# Autodesk Inventor assembly: Clamp-On Single Stage Gearbox
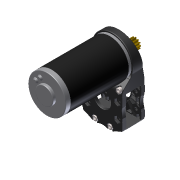
[picture p0: Inventor's stored thumbnail of the model, 180x180]
Saved by Autodesk Inventor 2015 (Build 190159000, 159)
## iProperties
Created: 2014-12-18
Part Number: Clamp-On Single Stage Gearbox
Document SubType Name: Assembly
Designer: Nemo
Author: Nemo
## Documents named in this file (8)
- H:\Nemo\Documents\Robotics\CAD Files\COTS Parts\Gearboxes\VexPro\Clamp-On Single Stage Gearbox.iam
- H:\Nemo\Documents\Robotics\CAD Files\COTS Parts\Gearboxes\VexPro\Components\Clamp-On Single Stage Gearbox motor side.ipt
- H:\Nemo\Documents\Robotics\CAD Files\COTS Parts\Gearboxes\VexPro\Components\Clamp-On Single Stage Gearbox gear side.ipt
- H:\Nemo\Documents\Robotics\CAD Files\COTS Parts\Fasteners\10-32\10-32 locknut.ipt
- H:\Nemo\Documents\Robotics\CAD Files\COTS Parts\Fasteners\10-32\10-32 SHCS x1375.ipt
- H:\Nemo\Documents\Robotics\CAD Files\COTS Parts\Motors\CIM motor.ipt
- H:\Nemo\Documents\Robotics\CAD Files\COTS Parts\Gears\Gear 20dp 10mm key 12T Vex.ipt
- H:\Nemo\Documents\Robotics\CAD Files\COTS Parts\Fasteners\10-32\10-32 SHCS x625.ipt
## Components (14 placed, 7 different names)
1. Clamp-On Single Stage Gearbox motor side:1 — Mate:6, Flush:1, Mate:7, Flush:3, Insert:9, Mate:8, Insert:10, Insert:11, Insert:12, Insert:13, Insert:14, Insert:15, Flush:4
2. Clamp-On Single Stage Gearbox gear side:1 — Insert:5, Insert:6, Insert:7, Insert:8, Mate:6, Flush:2, Mate:7
3. 10-32 locknut:1 — Insert:12
4. 10-32 locknut:2 — Insert:13
5. 10-32 locknut:3 — Insert:14
6. 10-32 locknut:4 — Insert:15
7. 10-32 SHCS x1375:1 — Insert:5
8. 10-32 SHCS x1375:2 — Insert:6
9. 10-32 SHCS x1375:3 — Insert:7
10. 10-32 SHCS x1375:4 — Insert:8
11. CIM motor:1 — Mate:5, Angle:1, Insert:9, Mate:8
12. Gear 20dp 10mm key 12T Vex:1 — Mate:5, Angle:1
13. 10-32 SHCS x625:1 — Insert:11
14. 10-32 SHCS x625:2 — Insert:10
## Relationships (20: Insert 11, Mate 4, Flush 4, Angle 1)
- Insert:5: Clamp-On Single Stage Gearbox gear side:1 ↔ 10-32 SHCS x1375:1
- Insert:6: Clamp-On Single Stage Gearbox gear side:1 ↔ 10-32 SHCS x1375:2
- Insert:7: Clamp-On Single Stage Gearbox gear side:1 ↔ 10-32 SHCS x1375:3
- Insert:8: Clamp-On Single Stage Gearbox gear side:1 ↔ 10-32 SHCS x1375:4
- Mate:5: CIM motor:1 ↔ Gear 20dp 10mm key 12T Vex:1
- Angle:1 (0 deg): CIM motor:1 ↔ Gear 20dp 10mm key 12T Vex:1
- Mate:6: Clamp-On Single Stage Gearbox motor side:1 ↔ Clamp-On Single Stage Gearbox gear side:1
- Flush:1: Clamp-On Single Stage Gearbox motor side:1
- Flush:2: Clamp-On Single Stage Gearbox gear side:1
- Mate:7: Clamp-On Single Stage Gearbox motor side:1 ↔ Clamp-On Single Stage Gearbox gear side:1
- Flush:3 (12.7 mm): Clamp-On Single Stage Gearbox motor side:1
- Insert:9: Clamp-On Single Stage Gearbox motor side:1 ↔ CIM motor:1
- Mate:8: Clamp-On Single Stage Gearbox motor side:1 ↔ CIM motor:1
- Insert:10: Clamp-On Single Stage Gearbox motor side:1 ↔ 10-32 SHCS x625:2
- Insert:11: Clamp-On Single Stage Gearbox motor side:1 ↔ 10-32 SHCS x625:1
- Insert:12: Clamp-On Single Stage Gearbox motor side:1 ↔ 10-32 locknut:1
- Insert:13: Clamp-On Single Stage Gearbox motor side:1 ↔ 10-32 locknut:2
- Insert:14: Clamp-On Single Stage Gearbox motor side:1 ↔ 10-32 locknut:3
- Insert:15: Clamp-On Single Stage Gearbox motor side:1 ↔ 10-32 locknut:4
- Flush:4: Clamp-On Single Stage Gearbox motor side:1
